# Autodesk Inventor assembly: 3D model celeho depa
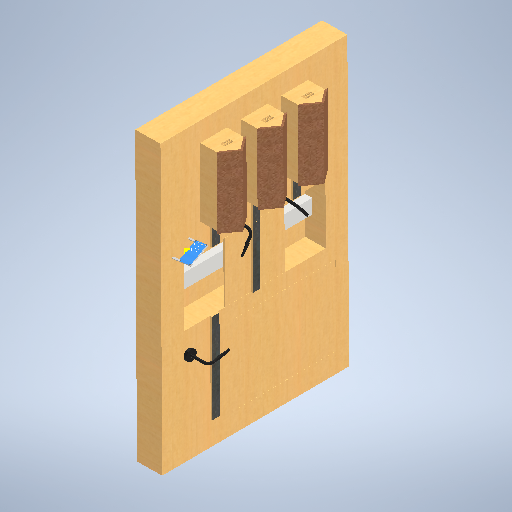
[picture p0: Inventor's stored thumbnail of the model, 512x512]
Saved by Autodesk Inventor 2025.1 (Build 291241000, 241)
## iProperties
Created: 2024-11-03
Part Number: 3D model celeho depa
Document SubType Name: Assembly
Designer: nelan
Author: nelan
## Documents named in this file (5)
- C:\Users\nelan\Documents\Nelca\Škola\_projekt\navrh\3D model celeho depa.iam
- C:\Users\nelan\Documents\Nelca\Škola\_projekt\navrh\3D cely.ipt
- C:\Users\nelan\Documents\Nelca\Škola\_projekt\navrh\prvni navrh garaze.ipt
- C:\Users\nelan\Documents\Nelca\Škola\_projekt\lampa ne moje.ipt
- C:\Users\nelan\Documents\Nelca\Škola\_projekt\navrh\displej ne muj.ipt
## Components (8 placed, 4 different names)
1. 3D cely:1 — Tuhé:1, Tuhé:2, Tuhé:3, Proti sobě:1
2. prvni navrh garaze:1 — Tuhé:1
3. prvni navrh garaze:2 — Tuhé:2
4. prvni navrh garaze:3 — Tuhé:3
5. lampa ne moje:1 — Proti sobě:1
6. lampa ne moje:2
7. lampa ne moje:3
8. displej ne muj:1
## Relationships (4: WeldJoint 3, Mate 1)
- Tuhé:1 [WeldJoint]: 3D cely:1 ↔ prvni navrh garaze:1
- Tuhé:2 [WeldJoint]: 3D cely:1 ↔ prvni navrh garaze:2
- Tuhé:3 [WeldJoint]: 3D cely:1 ↔ prvni navrh garaze:3
- Proti sobě:1 [Mate]: 3D cely:1 ↔ lampa ne moje:1
